# Autodesk Inventor assembly: Slider-Holder
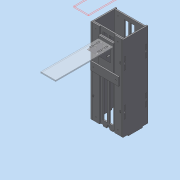
[picture p0: Inventor's stored thumbnail of the model, 180x180]
Saved by Autodesk Inventor 2016 SP1 (Build 200210100, 210)
## iProperties
Created: 2016-03-25
Part Number: Slider-Holder
Document SubType Name: Assembly
Designer: Mohamed A.
Author: Mohamed A.
## Documents named in this file (8)
- C:\Users\Mohamed\Documents\inventor\StemCellsPlatform\Laser Cut\Slider Holder\Slider-Holder.iam
- C:\Users\Mohamed\Documents\inventor\StemCellsPlatform\Laser Cut\Slider Holder\bed.ipt
- C:\Users\Mohamed\Documents\inventor\StemCellsPlatform\Laser Cut\Slider Holder\angle.ipt
- C:\Users\Mohamed\Documents\inventor\StemCellsPlatform\Laser Cut\Slider Holder\bed-axis.ipt
- C:\Users\Mohamed\Documents\inventor\StemCellsPlatform\Laser Cut\Slider Holder\axis-holder_front-front.ipt
- C:\Users\Mohamed\Documents\inventor\StemCellsPlatform\Laser Cut\Slider Holder\axis-holder_front-back.ipt
- C:\Users\Mohamed\Documents\inventor\StemCellsPlatform\Laser Cut\Slider Holder\axis-holder_plate.ipt
- C:\Users\Mohamed\Documents\inventor\StemCellsPlatform\Laser Cut\Slider Holder\slider-holder_side.ipt
## Components (11 placed, 7 different names)
1. bed:1 — Mate:1, Flush:1, Flush:2, Mate:2, Mate:3, Mate:4, Mate:5
2. angle:1 — Flush:2, Mate:2, Mate:3, Mate:7, Mate:8
3. angle:2 — Flush:1, Mate:4, Mate:5
4. bed-axis:1 — Mate:1, Mate:6, Flush:3, Flush:4, Mate:13
5. bed-axis:2 — Mate:6, Mate:7, Mate:8, Flush:3, Flush:4, Mate:10, Mate:11
6. axis-holder_front-front:1 — Mate:9, Flush:5, Flush:6, Mate:11, Mate:12, Mate:14
7. axis-holder_front-back:1 — Mate:9, Flush:5, Flush:6, Mate:10, Flush:7, Flush:8, Mate:15, Flush:9
8. axis-holder_plate:1 — Mate:12, Mate:13, Mate:14
9. axis-holder_front-back:2 — Flush:7, Flush:8, Mate:15, Flush:10, Mate:16, Flush:11, Flush:12, Mate:17
10. slider-holder_side:1 — Flush:9, Flush:10, Mate:16
11. slider-holder_side:2 — Flush:11, Flush:12, Mate:17
## Relationships (29: Mate 17, Flush 12)
- Mate:1: bed:1 ↔ bed-axis:1
- Flush:1: bed:1 ↔ angle:2
- Flush:2: bed:1 ↔ angle:1
- Mate:2: bed:1 ↔ angle:1
- Mate:3: bed:1 ↔ angle:1
- Mate:4: bed:1 ↔ angle:2
- Mate:5: bed:1 ↔ angle:2
- Mate:6: bed-axis:1 ↔ bed-axis:2
- Mate:7: angle:1 ↔ bed-axis:2
- Mate:8: angle:1 ↔ bed-axis:2
- Flush:3: bed-axis:1 ↔ bed-axis:2
- Flush:4: bed-axis:1 ↔ bed-axis:2
- Mate:9: axis-holder_front-front:1 ↔ axis-holder_front-back:1
- Flush:5: axis-holder_front-front:1 ↔ axis-holder_front-back:1
- Flush:6: axis-holder_front-front:1 ↔ axis-holder_front-back:1
- Mate:10: bed-axis:2 ↔ axis-holder_front-back:1
- Mate:11: bed-axis:2 ↔ axis-holder_front-front:1
- Mate:12: axis-holder_front-front:1 ↔ axis-holder_plate:1
- Mate:13: bed-axis:1 ↔ axis-holder_plate:1
- Mate:14: axis-holder_front-front:1 ↔ axis-holder_plate:1
- Flush:7: axis-holder_front-back:1 ↔ axis-holder_front-back:2
- Flush:8: axis-holder_front-back:1 ↔ axis-holder_front-back:2
- Mate:15 (50 mm): axis-holder_front-back:1 ↔ axis-holder_front-back:2
- Flush:9: axis-holder_front-back:1 ↔ slider-holder_side:1
- Flush:10: axis-holder_front-back:2 ↔ slider-holder_side:1
- Mate:16: axis-holder_front-back:2 ↔ slider-holder_side:1
- Flush:11: axis-holder_front-back:2 ↔ slider-holder_side:2
- Flush:12: axis-holder_front-back:2 ↔ slider-holder_side:2
- Mate:17: axis-holder_front-back:2 ↔ slider-holder_side:2
